# Autodesk Inventor assembly: cycloid_input_cam_assy.ipt
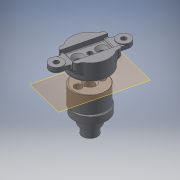
[picture p0: Inventor's stored thumbnail of the model, 180x180]
Saved by Autodesk Inventor 2019.4 (Build 234330000, 330)
## iProperties
Created: 2019-09-07
Part Number: cycloid_input_cam_assy.ipt
Document SubType Name: Assembly
Designer: cdi
Author: cdi
## Documents named in this file (3)
- D:\SynologyDrive\workspace_inventor\2019_06_19.MT4008_actuator\cycloid_gear_design_v2\cycloid_input_cam_assy.ipt.iam
- D:\SynologyDrive\workspace_inventor\2019_06_19.MT4008_actuator\cycloid_gear_design_v2\cycloid_input_cam_part1.ipt
- D:\SynologyDrive\workspace_inventor\2019_06_19.MT4008_actuator\cycloid_gear_design_v2\cycloid_input_cam_part2.ipt
## Components (2 placed, 2 different names)
1. cycloid_input_cam_part1:1 — Mate:1, Mate:2, Mate:3
2. cycloid_input_cam_part2:1 — Mate:1, Mate:2, Mate:3
## Relationships (3: Mate 3)
- Mate:1: cycloid_input_cam_part1:1 ↔ cycloid_input_cam_part2:1
- Mate:2: cycloid_input_cam_part1:1 ↔ cycloid_input_cam_part2:1
- Mate:3: cycloid_input_cam_part1:1 ↔ cycloid_input_cam_part2:1
